# Autodesk Inventor assembly: EL2-C-100
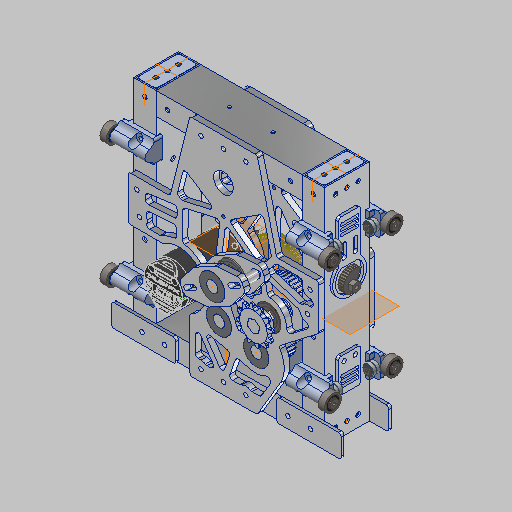
[picture p0: Inventor's stored thumbnail of the model, 512x512]
Saved by Autodesk Inventor 2023.5 (Build 275446000, 446)
## iProperties
Created: 2025-01-11
Part Number: EL2-C-100
Document SubType Name: Assembly
Designer: brand
Mass: 2629.85 g
Surface Area: 6187.7 cm^2
Volume: 981.459 cm^3
Author: brand
## Documents named in this file (11)
- C:\Users\slick\OneDrive\Desktop\2025-ReefScape---CAD\Elevator\EL2\EL2-C-100.iam
- C:\Users\slick\OneDrive\Desktop\2025-ReefScape---CAD\Elevator\EL2\EL2-C-001.ipt
- C:\Users\slick\OneDrive\Desktop\2025-ReefScape---CAD\Elevator\EL2\EL2-005.ipt
- C:\Users\slick\OneDrive\Desktop\2025-ReefScape---CAD\Elevator\EL2\EL2-C-005.ipt
- C:\Users\slick\OneDrive\Desktop\2025-ReefScape---CAD\COMMON PARTS\WCP Elevator parts\WCP-0323\WCP-0323.iam
- C:\Users\slick\OneDrive\Desktop\2025-ReefScape---CAD\Elevator\EL2-CGB\EL2-CGB-100.iam
- C:\Users\slick\OneDrive\Desktop\2025-ReefScape---CAD\Elevator\EL2\EL2-016.ipt
- C:\Users\slick\OneDrive\Desktop\2025-ReefScape---CAD\COMMON PARTS\WCP\WCP-0882.ipt
- C:\Users\slick\OneDrive\Desktop\2025-ReefScape---CAD\Elevator\EL2\EL2-019.ipt
- C:\Users\slick\OneDrive\Desktop\2025-ReefScape---CAD\Elevator\EL2\EL2-C-006.ipt
- C:\Users\slick\OneDrive\Desktop\2025-ReefScape---CAD\STEP files\sen36005_3d_model\sen36005_3d_model.iam
## Components (28 placed, 10 different names)
1. EL2-C-001:1 — Flush:4, Flush:8, Mate:10, Flush:9, Flush:11, Symmetry:2, Insert:53, Insert:55, Insert:57, Insert:59, Insert:76, Insert:77
2. EL2-C-005:2 — Insert:2, Angle:2, Flush:4, Mate:10, Insert:15, Insert:18, Insert:21, Insert:25, Insert:26, Insert:27, Mate:11, Insert:42, Insert:43, Symmetry:1, Insert:45, Insert:46, Insert:47, Insert:48, Insert:58, Insert:60, Insert:67, Insert:68, Mate:20, Insert:70, Insert:71, Insert:75
3. EL2-C-005:1 — Insert:8, Insert:10, Insert:32, Insert:33, Mate:12, Flush:12, Insert:34, Insert:37, Insert:38, Insert:39, Insert:40, Insert:41, Symmetry:1, Insert:49, Insert:50, Insert:54, Insert:56, Mate:19, Insert:65, Insert:66, Mate:21, Insert:72, Insert:73, Insert:74
4. EL2-C-001:4 — Flush:10, Flush:11, Mate:11, Mate:12, Flush:12, Symmetry:2, Insert:51, Insert:52
5. EL2-005:1 — Insert:2, Angle:2, Flush:9
6. EL2-005:2 — Insert:8, Flush:8
7. EL2-005:3 — Insert:10, Flush:10, Insert:32, Insert:33
8. EL2-005:4 — Insert:42, Insert:43
9. WCP-0323:1 [sub-assembly] — Insert:34, Insert:49
10. WCP-0323:2 [sub-assembly] — Insert:40, Insert:41
11. WCP-0323:3 [sub-assembly] — Insert:38, Insert:39
12. WCP-0323:4 [sub-assembly] — Insert:25, Insert:27, Insert:46
13. WCP-0323:5 [sub-assembly] — Insert:18, Insert:26
14. WCP-0323:6 [sub-assembly] — Insert:15, Insert:48
15. WCP-0323:7 [sub-assembly] — Insert:21, Insert:45, Insert:47
16. WCP-0323:8 [sub-assembly] — Insert:37, Insert:50
17. EL2-CGB-100:1 [sub-assembly] — Insert:51, Insert:52
18. EL2-016:1 — Insert:53, Insert:54
19. EL2-016:2 — Insert:55, Insert:56
20. EL2-016:3 — Insert:57, Insert:58
21. EL2-016:4 — Insert:59, Insert:60
22. WCP-0882:1 — Insert:75
23. WCP-0882:2 — Insert:74
24. EL2-019:1 — Mate:19, Insert:65, Insert:66
25. EL2-019:2 — Insert:67, Insert:68
26. EL2-C-006:1 — Mate:20, Insert:70, Insert:71
27. EL2-C-006:2 — Mate:21, Insert:72, Insert:73
28. sen36005_3d_model:1 [sub-assembly] — Insert:76, Insert:77
## Relationships (64: Insert 47, Mate 8, Flush 6, Symmetry 2, Angle 1)
- Insert:2: EL2-C-005:2 ↔ EL2-005:1
- Angle:2 (0 deg): EL2-C-005:2 ↔ EL2-005:1
- Insert:8: EL2-C-005:1 ↔ EL2-005:2
- Insert:10: EL2-C-005:1 ↔ EL2-005:3
- Flush:4: EL2-C-001:1 ↔ EL2-C-005:2
- Flush:8: EL2-C-001:1 ↔ EL2-005:2
- Mate:10: EL2-C-001:1 ↔ EL2-C-005:2
- Flush:9: EL2-C-001:1 ↔ EL2-005:1
- Flush:10: EL2-C-001:4 ↔ EL2-005:3
- Flush:11: EL2-C-001:1 ↔ EL2-C-001:4
- Insert:15: EL2-C-005:2 ↔ WCP-0323:6
- Insert:18: EL2-C-005:2 ↔ WCP-0323:5
- Insert:21: EL2-C-005:2 ↔ WCP-0323:7
- Insert:25: EL2-C-005:2 ↔ WCP-0323:4
- Insert:26: EL2-C-005:2 ↔ WCP-0323:5
- Insert:27: EL2-C-005:2 ↔ WCP-0323:4
- Insert:32: EL2-C-005:1 ↔ EL2-005:3
- Insert:33: EL2-C-005:1 ↔ EL2-005:3
- Mate:11: EL2-C-005:2 ↔ EL2-C-001:4
- Mate:12: EL2-C-005:1 ↔ EL2-C-001:4
- Flush:12: EL2-C-005:1 ↔ EL2-C-001:4
- Insert:34: EL2-C-005:1 ↔ WCP-0323:1
- Insert:37: EL2-C-005:1 ↔ WCP-0323:8
- Insert:38: EL2-C-005:1 ↔ WCP-0323:3
- Insert:39: EL2-C-005:1 ↔ WCP-0323:3
- Insert:40: EL2-C-005:1 ↔ WCP-0323:2
- Insert:41: EL2-C-005:1 ↔ WCP-0323:2
- Insert:42: EL2-C-005:2 ↔ EL2-005:4
- Insert:43: EL2-C-005:2 ↔ EL2-005:4
- Symmetry:1: EL2-C-005:2 ↔ EL2-C-005:1
- Symmetry:2: EL2-C-001:1 ↔ EL2-C-001:4
- Mate:13
- Mate:14
- Insert:45: EL2-C-005:2 ↔ WCP-0323:7
- Insert:46: EL2-C-005:2 ↔ WCP-0323:4
- Insert:47: EL2-C-005:2 ↔ WCP-0323:7
- Insert:48: EL2-C-005:2 ↔ WCP-0323:6
- Insert:49: EL2-C-005:1 ↔ WCP-0323:1
- Insert:50: EL2-C-005:1 ↔ WCP-0323:8
- Insert:51: EL2-C-001:4 ↔ EL2-CGB-100:1
- Insert:52: EL2-C-001:4 ↔ EL2-CGB-100:1
- Insert:53: EL2-C-001:1 ↔ EL2-016:1
- Insert:54: EL2-C-005:1 ↔ EL2-016:1
- Insert:55: EL2-C-001:1 ↔ EL2-016:2
- Insert:56: EL2-C-005:1 ↔ EL2-016:2
- Insert:57: EL2-C-001:1 ↔ EL2-016:3
- Insert:58: EL2-C-005:2 ↔ EL2-016:3
- Insert:59: EL2-C-001:1 ↔ EL2-016:4
- Insert:60: EL2-C-005:2 ↔ EL2-016:4
- Mate:19: EL2-C-005:1 ↔ EL2-019:1
- Insert:65: EL2-C-005:1 ↔ EL2-019:1
- Insert:66: EL2-C-005:1 ↔ EL2-019:1
- Insert:67: EL2-C-005:2 ↔ EL2-019:2
- Insert:68: EL2-C-005:2 ↔ EL2-019:2
- Mate:20: EL2-C-005:2 ↔ EL2-C-006:1
- Insert:70: EL2-C-005:2 ↔ EL2-C-006:1
- Insert:71: EL2-C-005:2 ↔ EL2-C-006:1
- Mate:21: EL2-C-005:1 ↔ EL2-C-006:2
- Insert:72: EL2-C-005:1 ↔ EL2-C-006:2
- Insert:73: EL2-C-005:1 ↔ EL2-C-006:2
- Insert:74: EL2-C-005:1 ↔ WCP-0882:2
- Insert:75: EL2-C-005:2 ↔ WCP-0882:1
- Insert:76: EL2-C-001:1 ↔ sen36005_3d_model:1
- Insert:77: EL2-C-001:1 ↔ sen36005_3d_model:1
